# Autodesk Inventor assembly: simulink
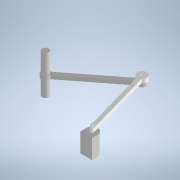
[picture p0: Inventor's stored thumbnail of the model, 180x180]
Saved by Autodesk Inventor 2021 (Build 250183000, 183)
## iProperties
Created: 2022-10-24
Part Number: simulink
Document SubType Name: Assembly
Designer: ivanm
Author: ivanm
## Documents named in this file (5)
- D:\UNAL\2022-2S\Servomecanismos\Proyecto Academico\Servomecanismo2R-main\Servomecanismo2R\INVENTOR\simulink.iam
- D:\UNAL\2022-2S\Servomecanismos\Proyecto Academico\Servomecanismo2R-main\Servomecanismo2R\INVENTOR\bancada.ipt
- D:\UNAL\2022-2S\Servomecanismos\Proyecto Academico\Servomecanismo2R-main\Servomecanismo2R\INVENTOR\eslabon1.ipt
- D:\UNAL\2022-2S\Servomecanismos\Proyecto Academico\Servomecanismo2R-main\Servomecanismo2R\INVENTOR\eslabon2.ipt
- D:\UNAL\2022-2S\Servomecanismos\Proyecto Academico\Marcador.ipt
## Components (4 placed, 4 different names)
1. bancada:1 — De rotación:1
2. eslabon1:1 — De rotación:1, Rotational:2
3. eslabon2:1 — Rotational:2, Rigid:1
4. Marcador:1 — Rigid:1
## Relationships (3: RevoluteJoint 2, WeldJoint 1)
- De rotación:1 [RevoluteJoint]: bancada:1 ↔ eslabon1:1
- Rotational:2 [RevoluteJoint] (8 mm): eslabon1:1 ↔ eslabon2:1
- Rigid:1 [WeldJoint]: eslabon2:1 ↔ Marcador:1
